# Autodesk Inventor assembly: Plate pulley
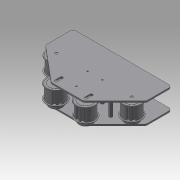
[picture p0: Inventor's stored thumbnail of the model, 180x180]
Saved by Autodesk Inventor 2016 (Build 200138000, 138)
## iProperties
Created: 2015-10-10
Part Number: Plate pulley
Document SubType Name: Assembly
Designer: Delta
Author: Delta
## Documents named in this file (4)
- C:\Robotics\CAD\2015-16\custom cad parts\Plate pulley.iam
- C:\Robotics\CAD\2015-16\custom cad parts\track side panel V1.ipt
- C:\Robotics\CAD\2015-16\custom cad parts\wheel & axil.iam
- C:\Robotics\CAD\2015-16\custom cad parts\Hex standoff custom.ipt
## Components (11 placed, 3 different names)
1. track side panel V1:1 — Mate:1, Mate:2, Mate:3
2. track side panel V1:2 — Insert:1, Insert:2, Insert:3, Insert:4, Insert:5, Insert:6, Insert:7, Insert:8, Insert:9
3. wheel & axil:1 [sub-assembly] — Insert:2, Mate:1
4. wheel & axil:2 [sub-assembly] — Insert:3, Mate:2
5. wheel & axil:3 [sub-assembly] — Insert:1
6. wheel & axil:4 [sub-assembly] — Insert:4
7. Hex standoff custom:1 — Insert:6, Mate:3
8. Hex standoff custom:2 — Insert:7
9. Hex standoff custom:3 — Insert:8
10. Hex standoff custom:4 — Insert:5
11. Hex standoff custom:5 — Insert:9
## Relationships (12: Insert 9, Mate 3)
- Insert:1: track side panel V1:2 ↔ wheel & axil:3
- Insert:2: track side panel V1:2 ↔ wheel & axil:1
- Insert:3: track side panel V1:2 ↔ wheel & axil:2
- Insert:4: track side panel V1:2 ↔ wheel & axil:4
- Mate:1: track side panel V1:1 ↔ wheel & axil:1
- Insert:5: track side panel V1:2 ↔ Hex standoff custom:4
- Insert:6: track side panel V1:2 ↔ Hex standoff custom:1
- Insert:7: track side panel V1:2 ↔ Hex standoff custom:2
- Insert:8: track side panel V1:2 ↔ Hex standoff custom:3
- Insert:9: track side panel V1:2 ↔ Hex standoff custom:5
- Mate:2: track side panel V1:1 ↔ wheel & axil:2
- Mate:3: track side panel V1:1 ↔ Hex standoff custom:1
